# Autodesk Inventor assembly: EnsamblajePantalla
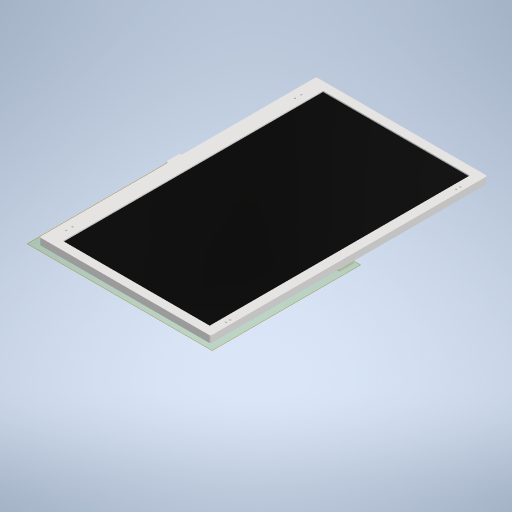
[picture p0: Inventor's stored thumbnail of the model, 512x512]
Saved by Autodesk Inventor 2023 (Build 270158000, 158)
## iProperties
Created: 2023-05-12
Part Number: EnsamblajePantalla
Document SubType Name: Assembly
Designer: sergi
Author: sergi
## Documents named in this file (10)
- C:\Users\sergi\OneDrive\Escritorio\Objetos 3d\pantalla\EnsamblajePantalla.iam
- C:\Users\sergi\OneDrive\Escritorio\Objetos 3d\pantalla\pantalla.ipt
- C:\Users\sergi\OneDrive\Escritorio\Objetos 3d\pantalla\UnionBrazoPantalla.ipt
- C:\Users\sergi\OneDrive\Escritorio\Objetos 3d\pantalla\TraseraPantallaDerecha.ipt
- C:\Users\sergi\OneDrive\Escritorio\Objetos 3d\pantalla\TraseraPantallaIzquierda.ipt
- C:\Users\sergi\OneDrive\Escritorio\Objetos 3d\pantalla\Union 4.ipt
- C:\Users\sergi\OneDrive\Escritorio\Objetos 3d\pantalla\Union abajo.ipt
- C:\Users\sergi\OneDrive\Escritorio\Objetos 3d\pantalla\MarcoDerecho.ipt
- C:\Users\sergi\OneDrive\Escritorio\Objetos 3d\pantalla\MarcoIzquierdo.ipt
- C:\Users\sergi\OneDrive\Escritorio\Objetos 3d\pantalla\soporte pantalla 2.ipt
## Components (9 placed, 9 different names)
1. pantalla:1 — Coincidencia:1, Coincidencia:2, Nivelación:1, Nivelación:2, Nivelación:3, Coincidencia:4, Coincidencia:5, Coincidencia:8
2. TraseraPantallaDerecha:1 — Coincidencia:2, Coincidencia:3, Nivelación:3, Coincidencia:7, Nivelación:6
3. TraseraPantallaIzquierda:1 — Coincidencia:1, Nivelación:1, Nivelación:2, Coincidencia:3, Coincidencia:13, Nivelación:5
4. MarcoDerecho:1 — Coincidencia:4, Coincidencia:6, Nivelación:4, Coincidencia:10, Coincidencia:14
5. MarcoIzquierdo:1 — Coincidencia:5, Coincidencia:6, Nivelación:4, Coincidencia:7, Coincidencia:8, Coincidencia:9, Coincidencia:11, Coincidencia:12, Coincidencia:15
6. UnionBrazoPantalla:1
7. Union abajo:1 — Coincidencia:9, Coincidencia:10, Coincidencia:11, Coincidencia:12
8. Union 4:1 — Coincidencia:13, Coincidencia:14, Coincidencia:15
9. soporte pantalla 2:1 — Nivelación:5, Nivelación:6
## Relationships (21: Mate 15, Flush 6)
- Coincidencia:1 [Mate]: pantalla:1 ↔ TraseraPantallaIzquierda:1
- Coincidencia:2 [Mate]: pantalla:1 ↔ TraseraPantallaDerecha:1
- Nivelación:1 [Flush]: pantalla:1 ↔ TraseraPantallaIzquierda:1
- Nivelación:2 [Flush]: pantalla:1 ↔ TraseraPantallaIzquierda:1
- Coincidencia:3 [Mate]: TraseraPantallaDerecha:1 ↔ TraseraPantallaIzquierda:1
- Nivelación:3 [Flush]: pantalla:1 ↔ TraseraPantallaDerecha:1
- Coincidencia:4 [Mate]: pantalla:1 ↔ MarcoDerecho:1
- Coincidencia:5 [Mate]: pantalla:1 ↔ MarcoIzquierdo:1
- Coincidencia:6 [Mate]: MarcoDerecho:1 ↔ MarcoIzquierdo:1
- Nivelación:4 [Flush]: MarcoDerecho:1 ↔ MarcoIzquierdo:1
- Coincidencia:7 [Mate] (0.5 mm): TraseraPantallaDerecha:1 ↔ MarcoIzquierdo:1
- Coincidencia:8 [Mate] (0.5 mm): pantalla:1 ↔ MarcoIzquierdo:1
- Coincidencia:9 [Mate]: MarcoIzquierdo:1 ↔ Union abajo:1
- Coincidencia:10 [Mate]: MarcoDerecho:1 ↔ Union abajo:1
- Coincidencia:11 [Mate]: MarcoIzquierdo:1 ↔ Union abajo:1
- Coincidencia:12 [Mate]: MarcoIzquierdo:1 ↔ Union abajo:1
- Coincidencia:13 [Mate]: TraseraPantallaIzquierda:1 ↔ Union 4:1
- Coincidencia:14 [Mate]: MarcoDerecho:1 ↔ Union 4:1
- Coincidencia:15 [Mate]: MarcoIzquierdo:1 ↔ Union 4:1
- Nivelación:5 [Flush]: TraseraPantallaIzquierda:1 ↔ soporte pantalla 2:1
- Nivelación:6 [Flush]: TraseraPantallaDerecha:1 ↔ soporte pantalla 2:1
